# Autodesk Inventor assembly: 6in Performance Hex Bore nitrile
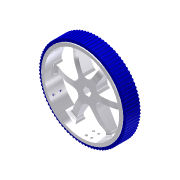
[picture p0: Inventor's stored thumbnail of the model, 180x180]
Saved by Autodesk Inventor 2011 (Build 150239000, 239)
## iProperties
Created: 2012-06-04
Part Number: 6in Performance Hex Bore nitrile
Document SubType Name: Assembly
Designer: Nemo
Author: Nemo
## Documents named in this file (3)
- H:\Nemo\Documents\Robotics\COTS Parts\Wheels\6in Performance Hex Bore nitrile.iam
- H:\Nemo\Documents\Robotics\COTS Parts\Wheels\Performance Wheel parts\6in Performance Hex.ipt
- H:\Nemo\Documents\Robotics\COTS Parts\Wheels\Tread\Nitrile Tread 6in.ipt
## Components (2 placed, 2 different names)
1. 6in Performance Hex:1 — Mate:1, Mate:2
2. Nitrile Tread 6in:1 — Mate:1, Mate:2
## Relationships (2: Mate 2)
- Mate:1: 6in Performance Hex:1 ↔ Nitrile Tread 6in:1
- Mate:2: 6in Performance Hex:1 ↔ Nitrile Tread 6in:1
